# Autodesk Inventor assembly: assembly
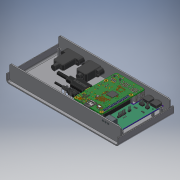
[picture p0: Inventor's stored thumbnail of the model, 180x180]
Saved by Autodesk Inventor 2017 (Build 210142000, 142)
## iProperties
Created: 2020-10-01
Part Number: assembly
Document SubType Name: Assembly
Designer: jferner
Author: jferner
## Documents named in this file (11)
- C:\dev\raspberry-pi-ir-hat\models3d\assembly.iam
- C:\dev\raspberry-pi-ir-hat\models3d\pcb\raspberry-pi-ir-hat.iam
- C:\dev\raspberry-pi-ir-hat\models3d\raspberry-pi-3\Raspberry Pi 3.iam
- C:\dev\raspberry-pi-ir-hat\models3d\case\case-bottom.ipt
- C:\dev\raspberry-pi-ir-hat\models3d\case\case-back.ipt
- C:\dev\raspberry-pi-ir-hat\models3d\case\case-front.ipt
- C:\dev\raspberry-pi-ir-hat\models3d\case\case-top.ipt
- C:\dev\raspberry-pi-ir-hat\models3d\USB-TypeB-Female-PanelMount\USB-TypeB-Female-PanelMount.iam
- C:\dev\raspberry-pi-ir-hat\models3d\USB-MicroPlug\Micro USB Plug.iam
- C:\dev\raspberry-pi-ir-hat\models3d\HDMI-Plug\HDMI.ipt
- C:\dev\raspberry-pi-ir-hat\models3d\HDMI-Female-PanelMount\HDMI-Female-PanelMount.iam
## Components (10 placed, 10 different names)
1. Raspberry Pi 3:1 [sub-assembly] — Mate:1, Flush:1, Flush:2, Mate:5, Mate:6, Mate:7, Mate:18, Mate:19, Mate:20, Mate:21, Mate:22, Mate:23
2. raspberry-pi-ir-hat:1 [sub-assembly] — Mate:1, Flush:1, Flush:2
3. case-bottom:1 — Mate:8, Mate:9, Mate:10, Mate:11, Mate:12, Mate:13
4. case-back:1 — Mate:5, Mate:6, Mate:7, Mate:11, Mate:12, Mate:13, Mate:14, Mate:15, Mate:16, Mate:17, Mate:25, Mate:26, Insert:1, Insert:2
5. case-front:1 — Mate:8, Mate:9, Mate:10
6. case-top:1 — Mate:14, Mate:15, Mate:16
7. USB-TypeB-Female-PanelMount:1 [sub-assembly] — Mate:17, Mate:25, Mate:26
8. Micro USB Plug:1 [sub-assembly] — Mate:18, Mate:19, Mate:20
9. HDMI:1 — Mate:21, Mate:22, Mate:23
10. HDMI-Female-PanelMount:1 [sub-assembly] — Insert:1, Insert:2
## Relationships (26: Mate 22, Flush 2, Insert 2)
- Mate:1: Raspberry Pi 3:1 ↔ raspberry-pi-ir-hat:1
- Flush:1: Raspberry Pi 3:1 ↔ raspberry-pi-ir-hat:1
- Flush:2: Raspberry Pi 3:1 ↔ raspberry-pi-ir-hat:1
- Mate:5 (0.5 mm): Raspberry Pi 3:1 ↔ case-back:1
- Mate:6 (0.5 mm): Raspberry Pi 3:1 ↔ case-back:1
- Mate:7 (0.5 mm): Raspberry Pi 3:1 ↔ case-back:1
- Mate:8: case-bottom:1 ↔ case-front:1
- Mate:9: case-bottom:1 ↔ case-front:1
- Mate:10: case-bottom:1 ↔ case-front:1
- Mate:11: case-bottom:1 ↔ case-back:1
- Mate:12: case-bottom:1 ↔ case-back:1
- Mate:13: case-bottom:1 ↔ case-back:1
- Mate:14: case-back:1 ↔ case-top:1
- Mate:15: case-back:1 ↔ case-top:1
- Mate:16: case-back:1 ↔ case-top:1
- Mate:17: case-back:1 ↔ USB-TypeB-Female-PanelMount:1
- Mate:18: Raspberry Pi 3:1 ↔ Micro USB Plug:1
- Mate:19: Raspberry Pi 3:1 ↔ Micro USB Plug:1
- Mate:20: Raspberry Pi 3:1 ↔ Micro USB Plug:1
- Mate:21: Raspberry Pi 3:1 ↔ HDMI:1
- Mate:22: Raspberry Pi 3:1 ↔ HDMI:1
- Mate:23: Raspberry Pi 3:1 ↔ HDMI:1
- Mate:25 (0.5 mm): case-back:1 ↔ USB-TypeB-Female-PanelMount:1
- Mate:26 (0.5 mm): case-back:1 ↔ USB-TypeB-Female-PanelMount:1
- Insert:1: case-back:1 ↔ HDMI-Female-PanelMount:1
- Insert:2: case-back:1 ↔ HDMI-Female-PanelMount:1
